# Autodesk Inventor assembly: trackingsolarpanel
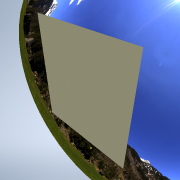
[picture p0: Inventor's stored thumbnail of the model, 180x180]
Saved by Autodesk Inventor 2020 (Build 240168000, 168)
## iProperties
Created: 2022-10-26
Part Number: trackingsolarpanel
Document SubType Name: Assembly
Designer: Admin
Author: Admin
## Documents named in this file (10)
- D:\4IEME - ANNEE INSA TOULOUSE\JUNCTIONX\Yettel\trackingsolarpanel.iam
- E:\PROJETHACKATHON\base motor.ipt
- D:\4IEME - ANNEE INSA TOULOUSE\JUNCTIONX\Yettel\Solide89.ipt
- D:\4IEME - ANNEE INSA TOULOUSE\JUNCTIONX\Yettel\Solide92.ipt
- D:\4IEME - ANNEE INSA TOULOUSE\JUNCTIONX\Yettel\solarpanelsmall.ipt
- D:\4IEME - ANNEE INSA TOULOUSE\JUNCTIONX\Yettel\Solide141.ipt
- D:\4IEME - ANNEE INSA TOULOUSE\JUNCTIONX\Yettel\Solide58.ipt
- D:\4IEME - ANNEE INSA TOULOUSE\JUNCTIONX\Yettel\Pièce3.ipt
- D:\4IEME - ANNEE INSA TOULOUSE\JUNCTIONX\breadboard-model-with-raspberry-pi-pico-1.snapshot.1\breadboard_case v1.iam
- D:\4IEME - ANNEE INSA TOULOUSE\JUNCTIONX\Yettel\maison-01.ipt
## Components (12 placed, 9 different names)
1. base motor:1 — Placage:1, Placage:2, Placage:3, Angle:8, Placage:16, Affleurement:2, Affleurement:3, Placage:19, Affleurement:4, Affleurement:5
2. Solide89:1 — Placage:1, Placage:2, Placage:3, Logement:1, Placage:10, Placage:11
3. Solide92:1 — Logement:1, Placage:4, Angle:7, Angle:6, Placage:5, Placage:6, Angle:9
4. Solide89:2 — Placage:4, Angle:7, Angle:6, Placage:5, Placage:6, Logement:2, Placage:12, Placage:13, Placage:14, Affleurement:1, Angle:10
5. Solide92:2 — Logement:2, Placage:17, Placage:18, Angle:10
6. solarpanelsmall:1 — Placage:17, Placage:18
7. Solide141:1 — Placage:10, Placage:11, Logement:3
8. Solide58:1 — Placage:12, Placage:13, Placage:15
9. Pièce3:1 — Logement:3, Angle:8
10. Pièce3:2 — Placage:14, Affleurement:1, Placage:15
11. breadboard_case v1:1 [sub-assembly] — Placage:16, Affleurement:2, Affleurement:3
12. maison-01:1 — Placage:19, Affleurement:4, Affleurement:5
## Relationships (29: Mate 16, Angle 5, Flush 5, Insert 3)
- Placage:1 [Mate]: base motor:1 ↔ Solide89:1
- Placage:2 [Mate] (10 mm): base motor:1 ↔ Solide89:1
- Placage:3 [Mate] (-32 mm): base motor:1 ↔ Solide89:1
- Logement:1 [Insert] (7.5 mm): Solide89:1 ↔ Solide92:1
- Placage:4 [Mate]: Solide92:1 ↔ Solide89:2
- Angle:7 (90 deg): Solide92:1 ↔ Solide89:2
- Angle:6 (180 deg): Solide92:1 ↔ Solide89:2
- Placage:5 [Mate]: Solide92:1 ↔ Solide89:2
- Placage:6 [Mate]: Solide92:1 ↔ Solide89:2
- Logement:2 [Insert] (7.5 mm): Solide89:2 ↔ Solide92:2
- Placage:10 [Mate]: Solide89:1 ↔ Solide141:1
- Placage:11 [Mate]: Solide89:1 ↔ Solide141:1
- Placage:12 [Mate]: Solide89:2 ↔ Solide58:1
- Placage:13 [Mate]: Solide89:2 ↔ Solide58:1
- Logement:3 [Insert]: Solide141:1 ↔ Pièce3:1
- Angle:8 (0 deg): base motor:1 ↔ Pièce3:1
- Placage:14 [Mate] (20 mm): Solide89:2 ↔ Pièce3:2
- Affleurement:1 [Flush] (-482 mm): Solide89:2 ↔ Pièce3:2
- Placage:15 [Mate] (-7.5 mm): Solide58:1 ↔ Pièce3:2
- Placage:16 [Mate]: base motor:1 ↔ breadboard_case v1:1
- Affleurement:2 [Flush] (69.804 mm): base motor:1 ↔ breadboard_case v1:1
- Affleurement:3 [Flush] (32.617 mm): base motor:1 ↔ breadboard_case v1:1
- Placage:17 [Mate]: Solide92:2 ↔ solarpanelsmall:1
- Placage:18 [Mate]: Solide92:2 ↔ solarpanelsmall:1
- Angle:9 (10.19 deg): Solide92:1
- Angle:10 (2.71 deg): Solide89:2 ↔ Solide92:2
- Placage:19 [Mate]: base motor:1 ↔ maison-01:1
- Affleurement:4 [Flush] (70 mm): base motor:1 ↔ maison-01:1
- Affleurement:5 [Flush] (200 mm): base motor:1 ↔ maison-01:1
